# Autodesk Inventor assembly: chaimber
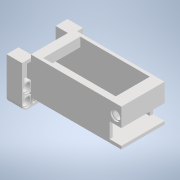
[picture p0: Inventor's stored thumbnail of the model, 180x180]
Saved by Autodesk Inventor 2021 (Build 250183000, 183)
## iProperties
Created: 2024-03-14
Part Number: chaimber
Document SubType Name: Assembly
Designer: 22hamfri
Author: 22hamfri
## Documents named in this file (3)
- C:\Users\22hamfri\Documents\School\Programmering\domino-bil\CAD\chaimber.iam
- C:\Users\22hamfri\Documents\School\Programmering\domino-bil\CAD\chaimber.ipt
- C:\Users\22hamfri\Documents\School\Programmering\domino-bil\CAD\chaimber-adapter.ipt
## Components (2 placed, 2 different names)
1. chaimber:1 — Rigid:1
2. chaimber-adapter:1 — Rigid:1
## Relationships (1: WeldJoint 1)
- Rigid:1 [WeldJoint]: chaimber:1 ↔ chaimber-adapter:1
